# Autodesk Inventor assembly: B_beam_V2
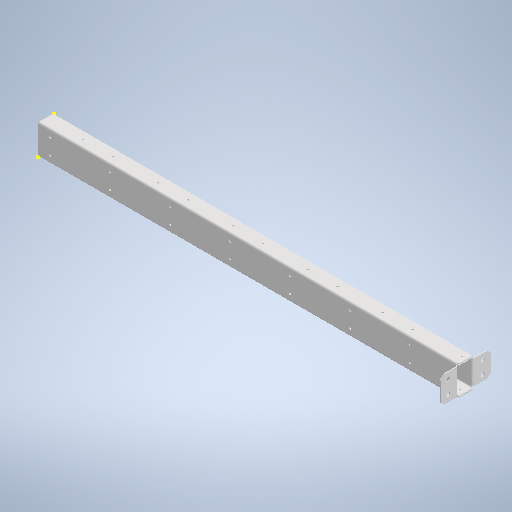
[picture p0: Inventor's stored thumbnail of the model, 512x512]
Saved by Autodesk Inventor 2025.1 (Build 291241000, 241)
## iProperties
Created: 2025-04-08
Part Number: B_beam_V2
Document SubType Name: Assembly
Designer: Caspe
Author: Caspe
## Documents named in this file (4)
- C:\Users\andpo\Documents\Anomaly_Detection\Mechanical_Project\Inventor_project\B_beam_V2.iam
- C:\Users\andpo\Documents\Anomaly_Detection\Mechanical_Project\Inventor_project\B_Beam.ipt
- C:\Users\andpo\Documents\Anomaly_Detection\Mechanical_Project\Inventor_project\B_beam_narrower.ipt
- C:\Users\andpo\Documents\Anomaly_Detection\Mechanical_Project\Inventor_project\Leg_press_parameters.xlsx
## Components (2 placed, 2 different names)
1. B_Beam:1 — Flush:1, Flush:2, Mate:5, Flush:3, Mate:6
2. B_beam_narrower:1 — Mate:5, Flush:3, Mate:6
## Relationships (7: Mate 4, Flush 3)
- Flush:1 (-25 mm): B_Beam:1
- Flush:2 (-25 mm): B_Beam:1
- Mate:3
- Mate:4
- Mate:5 (0.35 mm): B_Beam:1 ↔ B_beam_narrower:1
- Flush:3: B_Beam:1 ↔ B_beam_narrower:1
- Mate:6 (0.5 mm): B_Beam:1 ↔ B_beam_narrower:1
## Named parameters: A_length = 1000 mm, A_width = 46 mm, A_bend = 20 mm, A_connection_width = 40 mm, A_displacement = 500 mm, A_hole_height = 10 mm, A_hole_length = 40 mm, A_joint_diameter = 16 mm, A_height = 50 mm, A_joint_tolerance = 3 mm, l___________ = 0 mm, B_length = 700 mm, B_height = 50 mm, B_width = 50 mm, B_bend = 20 mm, B_connection_width = 40 mm, B_hole_height = 10 mm, B_hole_length = 40 mm, l__________ = 0 mm, C_length = 400 mm, C_width = 20 mm, C_height = 330 mm, l_________ = 0 mm, rivet_diameter = 3.35 mm, rivet_displacement = 250 mm, plate_thickness = 3 mm, l________ = 0 mm, B_hinge_holes_spacing = 50 mm, A_B_spacing = 2 mm, L_Piston_Bottom = 21 mm, L_Piston_Top = 25 mm, thin_plate = 1.5 mm
